# Autodesk Inventor assembly: 組合檔
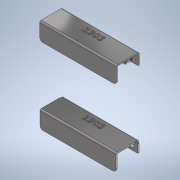
[picture p0: Inventor's stored thumbnail of the model, 180x180]
Saved by Autodesk Inventor 2020 (Build 240168000, 168)
## iProperties
Created: 2015-11-28
Part Number: 組合檔
Document SubType Name: Assembly
Designer: 設計製圖
Author: 設計製圖
## Documents named in this file (3)
- D:\資料庫\設計-3D Project\【May club 】\得利卡-車頂燈架\模型、圖面\22.01.05_設變 (未生產 )\差異.iam
- D:\資料庫\設計-3D Project\【May club 】\得利卡-車頂燈架\模型、圖面\22.01.05_設變 (未生產 )\ㄇ槽(#01.05)- 焊接組合.iam
- D:\資料庫\設計-3D Project\【May club 】\得利卡-車頂燈架\模型、圖面\短-車頂燈架-組合(#11.02)- 組合件2.iam
## Components (2 placed, 2 different names)
1. ㄇ槽(#01.05)- 焊接組合:1 [sub-assembly] — 齊平:2, 齊平:3
2. 短-車頂燈架-組合(#11.02)- 組合件2:1 [sub-assembly] — 齊平:2, 齊平:3
## Relationships (2: Flush 2)
- 齊平:2 [Flush]: ㄇ槽(#01.05)- 焊接組合:1 ↔ 短-車頂燈架-組合(#11.02)- 組合件2:1
- 齊平:3 [Flush]: ㄇ槽(#01.05)- 焊接組合:1 ↔ 短-車頂燈架-組合(#11.02)- 組合件2:1
